# Autodesk Inventor assembly: left wheel with clamping hub_MIR
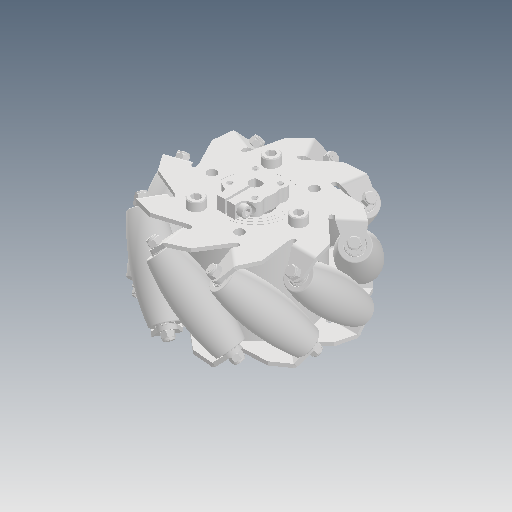
[picture p0: Inventor's stored thumbnail of the model, 512x512]
Saved by Autodesk Inventor 2020 (Build 240168000, 168)
## iProperties
Created: 2019-09-27
Part Number: left wheel with clamping hub_MIR
Document SubType Name: Assembly
Designer: ball
Author: ball
## Documents named in this file (3)
- C:\FTC\FTC8863CAD\2019 Robot\Mecanum Drive Train\left wheel with clamping hub_MIR.iam
- C:\FTC\FTC8863CAD\2019 Robot\Mecanum Drive Train\left wheel_MIR.iam
- C:\FTC\FTC8863CAD\Actobotics\545 parts\545618 assembly_MIR.ipt
## Components (3 placed, 2 different names)
1. left wheel_MIR:1 [sub-assembly] — Mate:6, Mate:2, Mate:7, Mate:4
2. 545618 assembly_MIR:1 — Mate:6, Mate:2, Flush:1
3. 545618 assembly_MIR:2 — Mate:7, Flush:1, Mate:4
## Relationships (5: Mate 4, Flush 1)
- Mate:6 (2.54 mm): left wheel_MIR:1 ↔ 545618 assembly_MIR:1
- Mate:2: left wheel_MIR:1 ↔ 545618 assembly_MIR:1
- Mate:7: left wheel_MIR:1 ↔ 545618 assembly_MIR:2
- Flush:1: 545618 assembly_MIR:1 ↔ 545618 assembly_MIR:2
- Mate:4: left wheel_MIR:1 ↔ 545618 assembly_MIR:2
